# Autodesk Inventor assembly: Part_dung
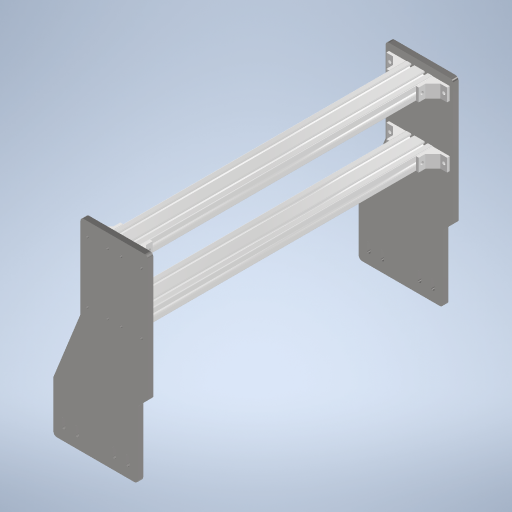
[picture p0: Inventor's stored thumbnail of the model, 512x512]
Saved by Autodesk Inventor 2023 (Build 270158000, 158)
## iProperties
Created: 2025-04-17
Part Number: Part_dung
Document SubType Name: Assembly
Designer: huyqu
Author: huyqu
## Documents named in this file (5)
- E:\TAI LIEU\Final_Project\DONE\CoCauTrucZ\Part_dung.iam
- E:\TAI LIEU\Final_Project\DONE\CoCauTrucZ\PA1.ipt
- E:\TAI LIEU\Final_Project\DONE\CoCauTrucZ\Alu_Profile_40x80x300\Alu_Profile_40x80x300-02.ipt
- E:\TAI LIEU\Final_Project\DONE\CoCauTrucZ\Alu_Profile_40x80x300.ipt
- E:\TAI LIEU\Final_Project\DONE\CoCauTrucZ\KeNhom40.ipt
## Components (12 placed, 3 different names)
1. PA1:1 — Mate:1, Flush:1, Flush:2, Mate:2, Flush:3, Flush:4, Mate:3, Flush:5, Flush:6, Mate:12, Mate:13, Mate:14, Mate:15, Mate:16, Mate:17, Mate:18, Mate:19
2. PA1:2 — Mate:1, Flush:1, Flush:2, Mate:4, Mate:5, Mate:6, Mate:7, Mate:8, Mate:9, Mate:10, Mate:11
3. Alu_Profile_40x80x300-02:1 — Mate:3, Flush:5, Flush:6
4. Alu_Profile_40x80x300-02:2 — Mate:2, Flush:3, Flush:4
5. KeNhom40:1 — Mate:12, Mate:13
6. KeNhom40:2 — Mate:14, Mate:15
7. KeNhom40:3 — Mate:16, Mate:17
8. KeNhom40:4 — Mate:18, Mate:19
9. KeNhom40:5 — Mate:4, Mate:5
10. KeNhom40:6 — Mate:6, Mate:7
11. KeNhom40:7 — Mate:8, Mate:9
12. KeNhom40:8 — Mate:10, Mate:11
## Relationships (25: Mate 19, Flush 6)
- Mate:1 (888 mm): PA1:1 ↔ PA1:2
- Flush:1: PA1:1 ↔ PA1:2
- Flush:2: PA1:1 ↔ PA1:2
- Mate:2: PA1:1 ↔ Alu_Profile_40x80x300-02:2
- Flush:3 (60 mm): PA1:1 ↔ Alu_Profile_40x80x300-02:2
- Flush:4 (20 mm): PA1:1 ↔ Alu_Profile_40x80x300-02:2
- Mate:3: PA1:1 ↔ Alu_Profile_40x80x300-02:1
- Flush:5 (60 mm): PA1:1 ↔ Alu_Profile_40x80x300-02:1
- Flush:6 (200 mm): PA1:1 ↔ Alu_Profile_40x80x300-02:1
- Mate:4: PA1:2 ↔ KeNhom40:5
- Mate:5: PA1:2 ↔ KeNhom40:5
- Mate:6: PA1:2 ↔ KeNhom40:6
- Mate:7: PA1:2 ↔ KeNhom40:6
- Mate:8: PA1:2 ↔ KeNhom40:7
- Mate:9: PA1:2 ↔ KeNhom40:7
- Mate:10: PA1:2 ↔ KeNhom40:8
- Mate:11: PA1:2 ↔ KeNhom40:8
- Mate:12: PA1:1 ↔ KeNhom40:1
- Mate:13: PA1:1 ↔ KeNhom40:1
- Mate:14: PA1:1 ↔ KeNhom40:2
- Mate:15: PA1:1 ↔ KeNhom40:2
- Mate:16: PA1:1 ↔ KeNhom40:3
- Mate:17: PA1:1 ↔ KeNhom40:3
- Mate:18: PA1:1 ↔ KeNhom40:4
- Mate:19: PA1:1 ↔ KeNhom40:4
